# Autodesk Inventor assembly: motor
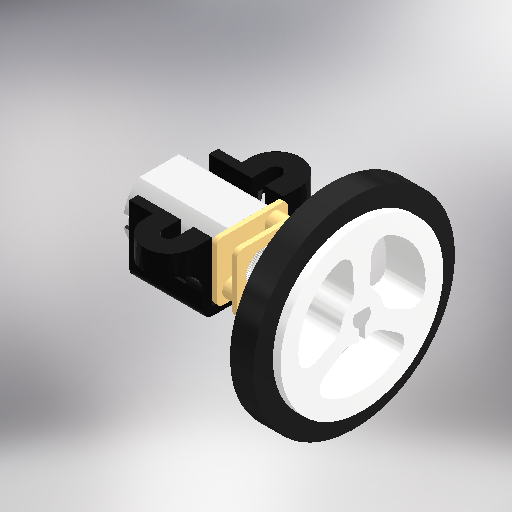
[picture p0: Inventor's stored thumbnail of the model, 512x512]
Saved by Autodesk Inventor 2025.2 (Build 292293000, 293)
## iProperties
Created: 2025-11-10
Part Number: motor
Document SubType Name: Assembly
Designer: ia088
Author: ia088
## Documents named in this file (4)
- C:\Users\ia088\OneDrive\Dokumen\Prak.Robotika\board fix\motor.iam
- C:\Users\ia088\OneDrive\Dokumen\Prak.Robotika\board fix\N20 DC Gear Motor\N20 DC Gear Motor\N20 DC Gear Motor.iam
- C:\Users\ia088\OneDrive\Dokumen\Prak.Robotika\board fix\N20 DC Gear Motor\motor mount-Body.ipt
- C:\Users\ia088\OneDrive\Dokumen\Prak.Robotika\board fix\n20-wheel-34mm-1.snapshot.1\Roda 34 mm\Roda 34 mm\Roda 34 mm.ipt
## Components (3 placed, 3 different names)
1. N20 DC Gear Motor:1 [sub-assembly] — Mate:1, Mate:2, Mate:3, Mate:4, Mate:5, Mate:6, Flush:1
2. motor mount-Body:1 — Mate:1, Mate:2, Mate:3, Mate:4
3. Roda 34 mm:1 — Mate:5, Mate:6, Flush:1
## Relationships (7: Mate 6, Flush 1)
- Mate:1: N20 DC Gear Motor:1 ↔ motor mount-Body:1
- Mate:2: N20 DC Gear Motor:1 ↔ motor mount-Body:1
- Mate:3: N20 DC Gear Motor:1 ↔ motor mount-Body:1
- Mate:4: N20 DC Gear Motor:1 ↔ motor mount-Body:1
- Mate:5: N20 DC Gear Motor:1 ↔ Roda 34 mm:1
- Mate:6: N20 DC Gear Motor:1 ↔ Roda 34 mm:1
- Flush:1: N20 DC Gear Motor:1 ↔ Roda 34 mm:1
